# Autodesk Inventor assembly: 200-03-BOGIE-CONNECTOR-ASM
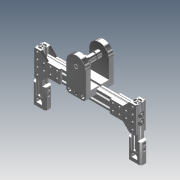
[picture p0: Inventor's stored thumbnail of the model, 180x180]
Saved by Autodesk Inventor 2018.2 (Build 222227000, 227)
## iProperties
Manager: feesmrt
Company: FRANCOR
Created: 2017-12-19
Part Number: 200-03-BOGIE-CONNECTOR-ASM
Project: Rescue Robot
Cost Center: -
Material: Generisch
Document SubType Name: Assembly
Designer: feesmrt
Engineer: feesmrt
Authority: feesmrt
Description: Bogie Connector
Stock Number: 200-03-BOGIE-CONNECTOR-ASM-L
Subject: Rescue Robot
Author: feesmrt
Revision Number: 1
Title: Bogie Connector
## Documents named in this file (5)
- D:\Programmierung\FRANC0R\CAD\02-Rocker-Bogie-Robot\200-ROCKER-BOGIE\200-03-BOGIE-CONNECTOR-ASM.iam
- D:\Programmierung\FRANC0R\CAD\02-Rocker-Bogie-Robot\200-ROCKER-BOGIE\200-40-BOGIE-CONNECTOR\200-40-BOGIE-CONNECTOR-ASM-01.iam
- D:\Programmierung\FRANC0R\CAD\02-Rocker-Bogie-Robot\200-ROCKER-BOGIE\200-50-WHEEL-CONNECTOR\200-50-WHEEL-CONNECTOR-20MM-ASM-01.iam
- D:\Programmierung\FRANC0R\CAD\02-Rocker-Bogie-Robot\900-COMPONENTS\900-40-SCREWS\900-40-SCREWS-DIN7984_M6x30.ipt
- D:\Programmierung\FRANC0R\CAD\02-Rocker-Bogie-Robot\900-COMPONENTS\900-80-WASHERS\900-80-WASHERS-DIN9021-M6.ipt
## Components (11 placed, 4 different names)
1. 200-40-BOGIE-CONNECTOR-ASM-01:1 [sub-assembly] — Passend:1, Fluchtend:1, Passend:2, Fluchtend:2, Passend:3, Passend:4, Passend:7, Passend:9, Passend:11, Passend:12, Passend:15, Passend:18, Passend:19, Passend:20
2. 200-50-WHEEL-CONNECTOR-20MM-ASM-01:1 [sub-assembly] — Passend:1, Fluchtend:1, Passend:2
3. 200-50-WHEEL-CONNECTOR-20MM-ASM-01:2 [sub-assembly] — Fluchtend:2, Passend:3, Passend:4
4. 900-40-SCREWS-DIN7984_M6x30:1 — Passend:5, Passend:8, Passend:9
5. 900-40-SCREWS-DIN7984_M6x30:2 — Passend:6, Passend:10, Passend:11
6. 900-40-SCREWS-DIN7984_M6x30:3 — Passend:13, Passend:16, Passend:19
7. 900-40-SCREWS-DIN7984_M6x30:4 — Passend:14, Passend:17, Passend:20
8. 900-80-WASHERS-DIN9021-M6:1 — Passend:5, Passend:7, Passend:8
9. 900-80-WASHERS-DIN9021-M6:2 — Passend:6, Passend:10, Passend:12
10. 900-80-WASHERS-DIN9021-M6:3 — Passend:13, Passend:15, Passend:16
11. 900-80-WASHERS-DIN9021-M6:4 — Passend:14, Passend:17, Passend:18
## Relationships (22: Mate 20, Flush 2)
- Passend:1 [Mate]: 200-40-BOGIE-CONNECTOR-ASM-01:1 ↔ 200-50-WHEEL-CONNECTOR-20MM-ASM-01:1
- Fluchtend:1 [Flush]: 200-40-BOGIE-CONNECTOR-ASM-01:1 ↔ 200-50-WHEEL-CONNECTOR-20MM-ASM-01:1
- Passend:2 [Mate]: 200-40-BOGIE-CONNECTOR-ASM-01:1 ↔ 200-50-WHEEL-CONNECTOR-20MM-ASM-01:1
- Fluchtend:2 [Flush]: 200-40-BOGIE-CONNECTOR-ASM-01:1 ↔ 200-50-WHEEL-CONNECTOR-20MM-ASM-01:2
- Passend:3 [Mate]: 200-40-BOGIE-CONNECTOR-ASM-01:1 ↔ 200-50-WHEEL-CONNECTOR-20MM-ASM-01:2
- Passend:4 [Mate]: 200-40-BOGIE-CONNECTOR-ASM-01:1 ↔ 200-50-WHEEL-CONNECTOR-20MM-ASM-01:2
- Passend:5 [Mate]: 900-40-SCREWS-DIN7984_M6x30:1 ↔ 900-80-WASHERS-DIN9021-M6:1
- Passend:6 [Mate]: 900-40-SCREWS-DIN7984_M6x30:2 ↔ 900-80-WASHERS-DIN9021-M6:2
- Passend:7 [Mate]: 200-40-BOGIE-CONNECTOR-ASM-01:1 ↔ 900-80-WASHERS-DIN9021-M6:1
- Passend:8 [Mate]: 900-40-SCREWS-DIN7984_M6x30:1 ↔ 900-80-WASHERS-DIN9021-M6:1
- Passend:9 [Mate]: 200-40-BOGIE-CONNECTOR-ASM-01:1 ↔ 900-40-SCREWS-DIN7984_M6x30:1
- Passend:10 [Mate]: 900-40-SCREWS-DIN7984_M6x30:2 ↔ 900-80-WASHERS-DIN9021-M6:2
- Passend:11 [Mate]: 200-40-BOGIE-CONNECTOR-ASM-01:1 ↔ 900-40-SCREWS-DIN7984_M6x30:2
- Passend:12 [Mate]: 200-40-BOGIE-CONNECTOR-ASM-01:1 ↔ 900-80-WASHERS-DIN9021-M6:2
- Passend:13 [Mate]: 900-40-SCREWS-DIN7984_M6x30:3 ↔ 900-80-WASHERS-DIN9021-M6:3
- Passend:14 [Mate]: 900-40-SCREWS-DIN7984_M6x30:4 ↔ 900-80-WASHERS-DIN9021-M6:4
- Passend:15 [Mate]: 200-40-BOGIE-CONNECTOR-ASM-01:1 ↔ 900-80-WASHERS-DIN9021-M6:3
- Passend:16 [Mate]: 900-40-SCREWS-DIN7984_M6x30:3 ↔ 900-80-WASHERS-DIN9021-M6:3
- Passend:17 [Mate]: 900-40-SCREWS-DIN7984_M6x30:4 ↔ 900-80-WASHERS-DIN9021-M6:4
- Passend:18 [Mate]: 200-40-BOGIE-CONNECTOR-ASM-01:1 ↔ 900-80-WASHERS-DIN9021-M6:4
- Passend:19 [Mate]: 200-40-BOGIE-CONNECTOR-ASM-01:1 ↔ 900-40-SCREWS-DIN7984_M6x30:3
- Passend:20 [Mate]: 200-40-BOGIE-CONNECTOR-ASM-01:1 ↔ 900-40-SCREWS-DIN7984_M6x30:4
